# Autodesk Inventor assembly: caja_nuevo
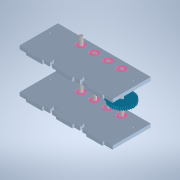
[picture p0: Inventor's stored thumbnail of the model, 180x180]
Saved by Autodesk Inventor 2022 (Build 260153000, 153)
## iProperties
Created: 2022-03-10
Part Number: caja_nuevo
Document SubType Name: Assembly
Designer: katha
Author: katha
## Documents named in this file (10)
- C:\Users\katha\OneDrive\Escritorio\Mini_Proyecto_Diseno\Diseno_18012\Modelo_MPD\caja_nuevo.iam
- C:\Users\katha\OneDrive\Escritorio\Mini_Proyecto_Diseno\Diseno_18012\Modelo_MPD\hombro_nuevo.ipt
- C:\Users\katha\OneDrive\Escritorio\Mini_Proyecto_Diseno\Diseno_18012\Modelo_MPD\engranaje10.ipt
- C:\Users\katha\OneDrive\Escritorio\Mini_Proyecto_Diseno\Diseno_18012\Modelo_MPD\engranaje40.ipt
- C:\Users\katha\OneDrive\Escritorio\Mini_Proyecto_Diseno\Diseno_18012\Modelo_MPD\eje1_n.ipt
- C:\Users\katha\OneDrive\Escritorio\Mini_Proyecto_Diseno\Diseno_18012\Modelo_MPD\caja_2_Lateral.ipt
- C:\Users\katha\OneDrive\Escritorio\Mini_Proyecto_Diseno\Diseno_18012\Modelo_MPD\Rodamiento_Ejes.ipt
- C:\Users\katha\OneDrive\Escritorio\Mini_Proyecto_Diseno\Diseno_18012\Modelo_MPD\eje2_n.ipt
- C:\Users\katha\OneDrive\Escritorio\Mini_Proyecto_Diseno\Diseno_18012\Modelo_MPD\eje3_n.ipt
- C:\Users\katha\OneDrive\Escritorio\Mini_Proyecto_Diseno\Diseno_18012\Modelo_MPD\eje4_n.ipt
## Components (24 placed, 9 different names)
1. hombro_nuevo:1 — Flush:1, Flush:2, Mate:1, Mate:22, Mate:23, Mate:24
2. hombro_nuevo:6 — Flush:11, Flush:12, Mate:6
3. engranaje10:2 — Flush:11, Flush:12, Mate:6, Flush:34
4. engranaje40:3 — Flush:1, Flush:2, Mate:1
5. eje1_n:1 — Mate:20, Mate:21, Flush:24, Mate:22, Mate:23, Mate:24
6. caja_2_Lateral:1 — Flush:13, Mate:12, Flush:16, Mate:13, Mate:14, Mate:15, Flush:17, Flush:18, Flush:19
7. caja_2_Lateral:2 — Flush:13, Mate:16, Mate:17, Mate:18, Mate:19, Flush:20, Flush:21, Flush:22, Flush:23
8. Rodamiento_Ejes:1 — Mate:12, Flush:16, Mate:20, Mate:21, Flush:24
9. Rodamiento_Ejes:2 — Mate:13, Flush:17, Flush:26
10. Rodamiento_Ejes:3 — Mate:14, Flush:18, Flush:27
11. Rodamiento_Ejes:4 — Mate:15, Flush:19
12. Rodamiento_Ejes:5 — Mate:16, Flush:20
13. Rodamiento_Ejes:6 — Mate:17, Flush:21
14. Rodamiento_Ejes:7 — Mate:18, Flush:22
15. Rodamiento_Ejes:8 — Mate:19, Flush:23, Flush:28
16. eje2_n:1 — Flush:26, Mate:25, Mate:26, Mate:27
17. eje3_n:1 — Flush:27, Mate:34
18. eje4_n:1 — Flush:28
19. hombro_nuevo:7 — Mate:25, Mate:26, Mate:27, Mate:28, Mate:29
20. engranaje10:3 — Mate:28, Mate:29, Mate:30, Flush:33
21. engranaje40:4 — Mate:30, Mate:31, Flush:33, Mate:35
22. engranaje40:5 — Mate:31, Mate:32, Flush:31, Flush:32, Mate:35, Flush:34
23. engranaje10:5 — Mate:32, Mate:33, Flush:29, Flush:30, Flush:32
24. hombro_nuevo:8 — Mate:33, Flush:29, Flush:30, Flush:31, Mate:34
## Relationships (49: Mate 26, Flush 23)
- Flush:1: hombro_nuevo:1 ↔ engranaje40:3
- Flush:2: hombro_nuevo:1 ↔ engranaje40:3
- Mate:1: hombro_nuevo:1 ↔ engranaje40:3
- Flush:11: hombro_nuevo:6 ↔ engranaje10:2
- Flush:12: hombro_nuevo:6 ↔ engranaje10:2
- Mate:6: hombro_nuevo:6 ↔ engranaje10:2
- Flush:13: caja_2_Lateral:1 ↔ caja_2_Lateral:2
- Mate:12: caja_2_Lateral:1 ↔ Rodamiento_Ejes:1
- Flush:16 (0.1 mm): caja_2_Lateral:1 ↔ Rodamiento_Ejes:1
- Mate:13: caja_2_Lateral:1 ↔ Rodamiento_Ejes:2
- Mate:14: caja_2_Lateral:1 ↔ Rodamiento_Ejes:3
- Mate:15: caja_2_Lateral:1 ↔ Rodamiento_Ejes:4
- Mate:16: caja_2_Lateral:2 ↔ Rodamiento_Ejes:5
- Mate:17: caja_2_Lateral:2 ↔ Rodamiento_Ejes:6
- Mate:18: caja_2_Lateral:2 ↔ Rodamiento_Ejes:7
- Mate:19: caja_2_Lateral:2 ↔ Rodamiento_Ejes:8
- Flush:17 (0.1 mm): caja_2_Lateral:1 ↔ Rodamiento_Ejes:2
- Flush:18 (0.1 mm): caja_2_Lateral:1 ↔ Rodamiento_Ejes:3
- Flush:19 (0.1 mm): caja_2_Lateral:1 ↔ Rodamiento_Ejes:4
- Flush:20 (0.1 mm): caja_2_Lateral:2 ↔ Rodamiento_Ejes:5
- Flush:21 (0.1 mm): caja_2_Lateral:2 ↔ Rodamiento_Ejes:6
- Flush:22 (0.1 mm): caja_2_Lateral:2 ↔ Rodamiento_Ejes:7
- Flush:23 (0.1 mm): caja_2_Lateral:2 ↔ Rodamiento_Ejes:8
- Mate:20 (0.4 mm): eje1_n:1 ↔ Rodamiento_Ejes:1
- Mate:21 (0.4 mm): eje1_n:1 ↔ Rodamiento_Ejes:1
- Flush:24: eje1_n:1 ↔ Rodamiento_Ejes:1
- Flush:26: Rodamiento_Ejes:2 ↔ eje2_n:1
- Flush:27: Rodamiento_Ejes:3 ↔ eje3_n:1
- Flush:28: Rodamiento_Ejes:8 ↔ eje4_n:1
- Mate:22: hombro_nuevo:1 ↔ eje1_n:1
- Mate:23: hombro_nuevo:1 ↔ eje1_n:1
- Mate:24: hombro_nuevo:1 ↔ eje1_n:1
- Mate:25: eje2_n:1 ↔ hombro_nuevo:7
- Mate:26: eje2_n:1 ↔ hombro_nuevo:7
- Mate:27: eje2_n:1 ↔ hombro_nuevo:7
- Mate:28: hombro_nuevo:7 ↔ engranaje10:3
- Mate:29: hombro_nuevo:7 ↔ engranaje10:3
- Mate:30: engranaje10:3 ↔ engranaje40:4
- Mate:31 (0.2 mm): engranaje40:4 ↔ engranaje40:5
- Mate:32: engranaje40:5 ↔ engranaje10:5
- Mate:33: engranaje10:5 ↔ hombro_nuevo:8
- Flush:29: engranaje10:5 ↔ hombro_nuevo:8
- Flush:30: engranaje10:5 ↔ hombro_nuevo:8
- Flush:31: engranaje40:5 ↔ hombro_nuevo:8
- Flush:32: engranaje40:5 ↔ engranaje10:5
- Mate:34: eje3_n:1 ↔ hombro_nuevo:8
- Flush:33: engranaje10:3 ↔ engranaje40:4
- Mate:35 (0.2 mm): engranaje40:4 ↔ engranaje40:5
- Flush:34 (-0.4 mm): engranaje10:2 ↔ engranaje40:5
